# Autodesk Inventor assembly: Spike
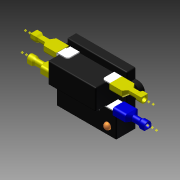
[picture p0: Inventor's stored thumbnail of the model, 180x180]
Saved by Autodesk Inventor 2011 (Build 150239000, 239)
## iProperties
Created: 2010-02-09
Part Number: Spike
Document SubType Name: Assembly
Designer: a
Author: a
## Documents named in this file (4)
- R:\2012\Inventor\vkop\All-Electrical\Spike.iam
- R:\2012\Inventor\vkop\All-Control-System\Control System_Innovation First_SPIKE-RELAY-H.ipt
- R:\2012\Inventor\vkop\All-Electrical\QuickDisconnect_Tyco_3-520408-2.ipt
- R:\2012\Inventor\vkop\All-Electrical\QuickDisconnect_Tyco_yellow.ipt
## Components (5 placed, 3 different names)
1. Control System_Innovation First_SPIKE-RELAY-H:1 — Mate:1, Flush:1, Mate:2, Mate:3, Mate:4, Mate:5, Mate:6, Flush:2, Mate:7, Mate:8, Mate:9, Mate:10
2. QuickDisconnect_Tyco_3-520408-2:1 — Mate:1, Flush:1, Mate:2
3. QuickDisconnect_Tyco_yellow:1 — Mate:6, Flush:2, Mate:10
4. QuickDisconnect_Tyco_yellow:2 — Mate:7, Mate:8, Mate:9
5. QuickDisconnect_Tyco_yellow:3 — Mate:3, Mate:4, Mate:5
## Relationships (12: Mate 10, Flush 2)
- Mate:1: Control System_Innovation First_SPIKE-RELAY-H:1 ↔ QuickDisconnect_Tyco_3-520408-2:1
- Flush:1: Control System_Innovation First_SPIKE-RELAY-H:1 ↔ QuickDisconnect_Tyco_3-520408-2:1
- Mate:2: Control System_Innovation First_SPIKE-RELAY-H:1 ↔ QuickDisconnect_Tyco_3-520408-2:1
- Mate:3: Control System_Innovation First_SPIKE-RELAY-H:1 ↔ QuickDisconnect_Tyco_yellow:3
- Mate:4: Control System_Innovation First_SPIKE-RELAY-H:1 ↔ QuickDisconnect_Tyco_yellow:3
- Mate:5: Control System_Innovation First_SPIKE-RELAY-H:1 ↔ QuickDisconnect_Tyco_yellow:3
- Mate:6: Control System_Innovation First_SPIKE-RELAY-H:1 ↔ QuickDisconnect_Tyco_yellow:1
- Flush:2: Control System_Innovation First_SPIKE-RELAY-H:1 ↔ QuickDisconnect_Tyco_yellow:1
- Mate:7: Control System_Innovation First_SPIKE-RELAY-H:1 ↔ QuickDisconnect_Tyco_yellow:2
- Mate:8: Control System_Innovation First_SPIKE-RELAY-H:1 ↔ QuickDisconnect_Tyco_yellow:2
- Mate:9: Control System_Innovation First_SPIKE-RELAY-H:1 ↔ QuickDisconnect_Tyco_yellow:2
- Mate:10: Control System_Innovation First_SPIKE-RELAY-H:1 ↔ QuickDisconnect_Tyco_yellow:1
